# Autodesk Inventor assembly: doorLockAssembly_V4
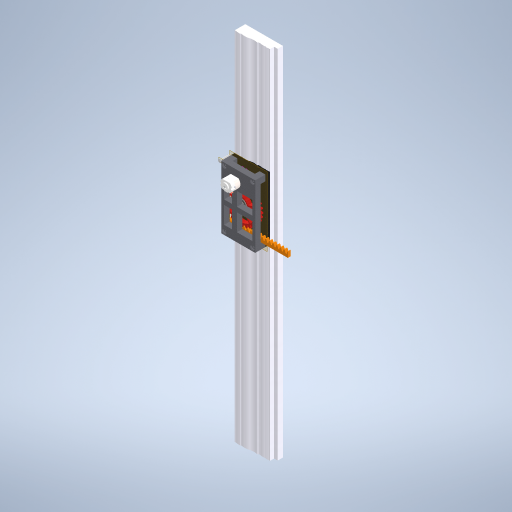
[picture p0: Inventor's stored thumbnail of the model, 512x512]
Saved by Autodesk Inventor 2023 (Build 270158000, 158)
## iProperties
Created: 2022-11-28
Part Number: doorLockAssembly_V4
Document SubType Name: Assembly
Designer: shrey
Author: shrey
## Documents named in this file (12)
- D:\Inventor Projects\Door Lock\V4\doorLockAssembly_V4.iam
- D:\Inventor Projects\Door Lock\V4\doorLockAssembly_V4\Design Accelerator\Spur Gears2.iam
- D:\Inventor Projects\Door Lock\V4\mouldingTestFitPiece.ipt
- D:\Inventor Projects\Door Lock\V4\moulding.ipt
- D:\Inventor Projects\Door Lock\V4\pinion_V4.ipt
- D:\Inventor Projects\Door Lock\V4\gear_V4.ipt
- D:\Inventor Projects\Door Lock\BallBearing_8x22x7mm.ipt
- D:\Inventor Projects\Door Lock\motor.ipt
- D:\Inventor Projects\Door Lock\V4\housingPlate.ipt
- D:\Inventor Projects\Door Lock\V3\rack_V3.ipt
- D:\Inventor Projects\headphone cable thing\housingFront.ipt
- D:\Inventor Projects\Door Lock\V4\screw.ipt
## Components (11 placed, 11 different names)
1. Spur Gears:1 [sub-assembly]
2. mouldingTestFitPiece:1 — Flush:1, Mate:1
3. moulding:1 — Mate:2, Mate:3, Flush:2
4. pinion_V4:1 — Flush:3, Mate:4
5. gear_V4:1 — Mate:10, Flush:8
6. BallBearing_8x22x7mm:1 — Flush:8
7. motor:1 — Flush:3, Mate:4
8. housingPlate:1 — Mate:7, Mate:8, Flush:5, Mate:10, Flush:10, Flush:11
9. rack_V3:1
10. housingFront:1 — Flush:11, Flush:12
11. screw:1 — Mate:12, Mate:13, Flush:9, Flush:10, Flush:12
## Relationships (18: Flush 9, Mate 9)
- Flush:1: mouldingTestFitPiece:1
- Mate:1: mouldingTestFitPiece:1
- Mate:2 (-18.749 mm): moulding:1
- Mate:3 (-58.171 mm): moulding:1
- Flush:2: moulding:1
- Flush:3: pinion_V4:1 ↔ motor:1
- Mate:4: pinion_V4:1 ↔ motor:1
- Mate:7: housingPlate:1
- Mate:8: housingPlate:1
- Flush:5: housingPlate:1
- Mate:10: gear_V4:1 ↔ housingPlate:1
- Flush:8: gear_V4:1 ↔ BallBearing_8x22x7mm:1
- Mate:12: screw:1
- Mate:13: screw:1
- Flush:9: screw:1
- Flush:10 (-3 mm): housingPlate:1 ↔ screw:1
- Flush:11: housingPlate:1 ↔ housingFront:1
- Flush:12: housingFront:1 ↔ screw:1
## Named parameters: t = 0.15 mm, bearingDepth = 8 mm
